# Autodesk Inventor assembly: 0905_bt_robot
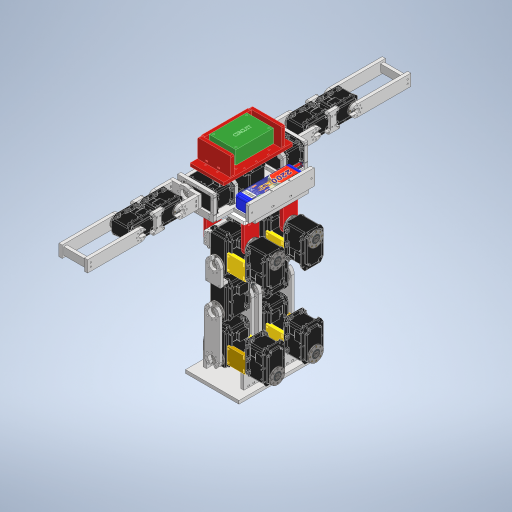
[picture p0: Inventor's stored thumbnail of the model, 512x512]
Saved by Autodesk Inventor 2024.3 (Build 283343000, 343)
## iProperties
Created: 2024-09-05
Part Number: 0905_bt_robot
Document SubType Name: Assembly
Designer: gretc
Author: gretc
## Documents named in this file (47)
- C:\Users\gretc\Desktop\inventor_part\예비인턴 격투로봇 설계 프로젝트\0905_bt_robot.iam
- C:\Users\gretc\Desktop\inventor_part\Motor_106.iam
- C:\Users\gretc\Desktop\inventor_part\Motor_64.iam
- C:\Users\gretc\Desktop\inventor_part\예비인턴 격투로봇 설계 프로젝트\_idle_adt.ipt
- C:\Users\gretc\Desktop\inventor_part\예비인턴 격투로봇 설계 프로젝트\_adle_adt_2.ipt
- C:\Users\gretc\Desktop\inventor_part\아이들러\64아이들러.iam
- C:\Users\gretc\Desktop\inventor_part\예비인턴 격투로봇 설계 프로젝트\_shim.ipt
- C:\Users\gretc\Desktop\inventor_part\예비인턴 격투로봇 설계 프로젝트\_foot.ipt
- C:\Users\gretc\Desktop\inventor_part\예비인턴 격투로봇 설계 프로젝트\_adle_adt_foot.ipt
- C:\Users\gretc\Desktop\inventor_part\예비인턴 격투로봇 설계 프로젝트\_foot_adt.ipt
- C:\Users\gretc\Desktop\inventor_part\예비인턴 격투로봇 설계 프로젝트\_108-64_adt.ipt
- C:\Users\gretc\Desktop\inventor_part\예비인턴 격투로봇 설계 프로젝트\_thigh.ipt
- C:\Users\gretc\Desktop\inventor_part\예비인턴 격투로봇 설계 프로젝트\_thigh_2.ipt
- C:\Users\gretc\Desktop\inventor_part\Motor_106_MIR.iam
- C:\Users\gretc\Desktop\inventor_part\Motor_64_MIR.iam
- C:\Users\gretc\Desktop\inventor_part\예비인턴 격투로봇 설계 프로젝트\_idle_adt_MIR.ipt
- C:\Users\gretc\Desktop\inventor_part\예비인턴 격투로봇 설계 프로젝트\_adle_adt_2_MIR.ipt
- C:\Users\gretc\Desktop\inventor_part\예비인턴 격투로봇 설계 프로젝트\_shim_MIR.ipt
- C:\Users\gretc\Desktop\inventor_part\예비인턴 격투로봇 설계 프로젝트\_foot_MIR.ipt
- C:\Users\gretc\Desktop\inventor_part\예비인턴 격투로봇 설계 프로젝트\_foot_adt_MIR.ipt
- C:\Users\gretc\Desktop\inventor_part\예비인턴 격투로봇 설계 프로젝트\_108-64_adt_MIR.ipt
- C:\Users\gretc\Desktop\inventor_part\예비인턴 격투로봇 설계 프로젝트\_thigh_MIR.ipt
- C:\Users\gretc\Desktop\inventor_part\예비인턴 격투로봇 설계 프로젝트\_thigh_2_MIR.ipt
- C:\Users\gretc\Desktop\inventor_part\아이들러\64아이들러_MIR2.iam
- C:\Users\gretc\Desktop\inventor_part\예비인턴 격투로봇 설계 프로젝트\_thigh_adt_body_MIR.ipt
- C:\Users\gretc\Desktop\inventor_part\혼\64-106Horn.ipt
- C:\Users\gretc\Desktop\inventor_part\다이나믹셀\MX-64T.ipt
- C:\Users\gretc\Desktop\inventor_part\Motor_28.iam
- C:\Users\gretc\Desktop\inventor_part\Motor_64_no_idle_ver.iam
- C:\Users\gretc\Desktop\inventor_part\예비인턴 격투로봇 설계 프로젝트\_arm_adt.ipt
- C:\Users\gretc\Desktop\inventor_part\예비인턴 격투로봇 설계 프로젝트\_armpit_adt_1.ipt
- C:\Users\gretc\Desktop\inventor_part\Power_Control_inventor\Enrichpower_2200mAh_11.1V_30C.ipt
- C:\Users\gretc\Desktop\inventor_part\예비인턴 격투로봇 설계 프로젝트\_hand_adt_ver_2_.ipt
- C:\Users\gretc\Desktop\inventor_part\예비인턴 격투로봇 설계 프로젝트\_fist_ver2_.ipt
- C:\Users\Public\Documents\Autodesk\Inventor 2024\_pelvis.ipt
- C:\Users\Public\Documents\Autodesk\Inventor 2024\_idle-pelvis_adt.ipt
- C:\Users\Public\Documents\Autodesk\Inventor 2024\_battery_adt.ipt
- C:\Users\Public\Documents\Autodesk\Inventor 2024\_battery_adt_2_.ipt
- C:\Users\Public\Documents\Autodesk\Inventor 2024\_newbody1.ipt
- C:\Users\Public\Documents\Autodesk\Inventor 2024\_face_froward_2.ipt
- C:\Users\Public\Documents\Autodesk\Inventor 2024\_body_side_ver2.ipt
- C:\Users\Public\Documents\Autodesk\Inventor 2024\head.iam
- C:\Users\Public\Documents\Autodesk\Inventor 2024\_inner.ipt
- C:\Users\Public\Documents\Autodesk\Inventor 2024\_arm_adt-ver2.ipt
- C:\Users\Public\Documents\Autodesk\Inventor 2024\_arm_pti.ipt
- C:\Users\gretc\Desktop\inventor_part\Power_Control_inventor\Circuit.ipt
- MX-106T+idle.ipt
## Components (95 placed, 45 different names)
1. Motor_106:1 [sub-assembly] — 메이트:1, 플러쉬:1, 플러쉬:2, 플러쉬:3, 플러쉬:5, 메이트:4, 메이트:6, 플러쉬:9, 플러쉬:11, 플러쉬:12, 메이트:24, 메이트:26, 메이트:29, 플러쉬:13, 삽입:3, 플러쉬:22, 메이트:38, 삽입:5, 삽입:6
2. Motor_106:2 [sub-assembly] — 플러쉬:3, 플러쉬:4, 플러쉬:5, 플러쉬:6, 메이트:3, 메이트:5, 메이트:6, 플러쉬:14, 삽입:2, 플러쉬:23, 삽입:9, 삽입:10
3. Motor_106:3 [sub-assembly] — 플러쉬:4, 플러쉬:6, 메이트:2, 메이트:5, 각도:1, 각도:2, 플러쉬:10, 메이트:8, 메이트:9, 메이트:10, 메이트:11, 삽입:11, 메이트:39, 삽입:12, 삽입:13, 삽입:22, 삽입:23
4. Motor_64:1 [sub-assembly] — 플러쉬:7, 플러쉬:8, 각도:1, 각도:2, 플러쉬:10, 메이트:8, 메이트:14, 메이트:15, 각도:5, 삽입:15
5. Motor_64:2 [sub-assembly] — 플러쉬:7, 플러쉬:8, 메이트:7, 플러쉬:9, 삽입:4, 플러쉬:20, 플러쉬:21
6. _idle_adt:1 — 플러쉬:11, 플러쉬:12, 메이트:30
7. _idle_adt:2 — 메이트:23, 메이트:25, 메이트:29
8. _adle_adt_2:1 — 플러쉬:13, 메이트:32, 삽입:1
9. 64아이들러:1 [sub-assembly] — 메이트:31, 삽입:1, 플러쉬:15, 플러쉬:16, 플러쉬:17, 메이트:33, 메이트:34, 플러쉬:18
10. _shim:1 — 플러쉬:14, 각도:3
11. _shim:2 — 삽입:2, 삽입:3
12. _foot:1 — 플러쉬:19, 플러쉬:26
13. _adle_adt_foot:1 — 플러쉬:15
14. _foot_adt:1 — 플러쉬:16, 플러쉬:17, 플러쉬:18, 각도:4
15. _foot_adt:2 — 삽입:4, 각도:4, 플러쉬:19
16. _108-64_adt:1 — 플러쉬:20, 플러쉬:21, 플러쉬:22
17. _108-64_adt:2 — 메이트:37, 삽입:5, 삽입:6
18. _thigh:1 — 플러쉬:23
19. _thigh_2:1
20. _thigh_2:2 — 삽입:7, 삽입:8
21. _thigh:2 — 삽입:7, 삽입:8, 삽입:9, 삽입:10
22. _108-64_adt:3 — 삽입:11, 메이트:39
23. _108-64_adt:4 — 삽입:12, 삽입:13
24. _foot_adt:4 — 각도:5, 삽입:15, 각도:14
25. 64아이들러:2 [sub-assembly] — 삽입:17, 메이트:40, 메이트:41, 삽입:118
26. _adle_adt_2:2 — 삽입:17, 삽입:18, 삽입:19, 삽입:20, 삽입:21
27. _idle_adt:3 — 삽입:18, 삽입:19, 삽입:22
28. _idle_adt:4 — 삽입:20, 삽입:21, 삽입:23
29. Motor_106_MIR:1 [sub-assembly] — 플러쉬:27, 플러쉬:28, 메이트:43, 메이트:44, 플러쉬:29, 플러쉬:30, 메이트:48, 플러쉬:34, 메이트:56, 메이트:57, 메이트:58, 메이트:61, 메이트:64, 메이트:65, 삽입:24, 메이트:70, 삽입:27, 삽입:28, 메이트:74
30. Motor_106_MIR:2 [sub-assembly] — 메이트:44, 플러쉬:29, 플러쉬:30, 메이트:45, 플러쉬:31, 플러쉬:32, 메이트:47, 메이트:68, 삽입:25, 메이트:75, 삽입:29, 삽입:30
31. Motor_106_MIR:3 [sub-assembly] — 메이트:45, 플러쉬:31, 플러쉬:32, 메이트:46, 메이트:49, 플러쉬:33, 각도:7, 각도:8, 메이트:51, 메이트:52, 메이트:53, 메이트:76, 삽입:33, 삽입:34, 삽입:35, 삽입:38, 삽입:41
32. Motor_64_MIR:1 [sub-assembly] — 메이트:49, 플러쉬:33, 각도:7, 각도:8, 플러쉬:35, 플러쉬:36, 메이트:54, 메이트:55, 삽입:36, 각도:11
33. Motor_64_MIR:2 [sub-assembly] — 플러쉬:34, 플러쉬:35, 플러쉬:36, 메이트:50, 삽입:26, 메이트:71, 메이트:72
34. _idle_adt_MIR:1 — 메이트:56, 메이트:57, 메이트:66
35. _idle_adt_MIR:2 — 메이트:58, 메이트:59, 메이트:62
36. _adle_adt_2_MIR:1 — 메이트:65, 메이트:67, 삽입:91
37. _shim_MIR:1 — 메이트:68, 각도:9
38. _shim_MIR:2 — 삽입:24, 삽입:25
39. _foot_MIR:1 — 메이트:69, 메이트:81
40. _foot_adt_MIR:1 — 메이트:144
41. _foot_adt_MIR:2 — 메이트:69, 삽입:26
42. _108-64_adt_MIR:1 — 메이트:70, 메이트:71, 메이트:72
43. _108-64_adt_MIR:2 — 삽입:27, 삽입:28, 메이트:73
44. _thigh_MIR:1 — 메이트:75
45. _thigh_2_MIR:1
46. _thigh_2_MIR:2 — 삽입:31, 삽입:32
47. _thigh_MIR:2 — 삽입:29, 삽입:30, 삽입:31, 삽입:32
48. _108-64_adt_MIR:3 — 메이트:76, 삽입:33
49. _108-64_adt_MIR:4 — 삽입:34, 삽입:35
50. _foot_adt_MIR:3 — 삽입:36, 각도:11, 플러쉬:102, 플러쉬:103, 플러쉬:104
51. 64아이들러_MIR2:1 [sub-assembly] — 삽입:37, 메이트:78, 메이트:79, 삽입:117
52. _adle_adt_2_MIR:2 — 삽입:37, 삽입:39, 삽입:40, 삽입:42, 삽입:43
53. _idle_adt_MIR:3 — 삽입:38, 삽입:39, 삽입:40
54. _idle_adt_MIR:4 — 삽입:41, 삽입:42, 삽입:43
55. 64아이들러:3 [sub-assembly] — 삽입:91, 메이트:143
56. MX-64T:1 — 삽입:119, 각도:15, 각도:16, 플러쉬:108, 플러쉬:109, 플러쉬:112, 플러쉬:113, 메이트:175, 메이트:176, 플러쉬:115, 플러쉬:116
57. 64-106Horn:1 — 삽입:119, 삽입:120, 플러쉬:107
58. _pelvis:1 — 플러쉬:102, 플러쉬:103, 플러쉬:104, 각도:15, 각도:16, 삽입:120, 각도:17
59. _thigh_adt_body_MIR:3 — 삽입:117, 각도:13
60. _thigh_adt_body_MIR:4 — 삽입:118, 각도:13, 각도:14
61. _idle-pelvis_adt:1 — 플러쉬:107
62. _armpit_adt_1:11 — 삽입:156, 삽입:157, 플러쉬:127
63. Motor_28:9 [sub-assembly] — 삽입:148, 삽입:149, 삽입:150, 삽입:153, 삽입:154, 삽입:155, 삽입:156, 삽입:157
64. Motor_28:10 [sub-assembly] — 삽입:144, 삽입:145, 삽입:146, 삽입:147, 삽입:151, 삽입:152, 삽입:158, 삽입:159
65. _arm_adt:9 — 삽입:150, 삽입:151, 삽입:152, 삽입:153
66. _arm_adt:10 — 삽입:146, 삽입:147, 삽입:148, 삽입:149
67. _armpit_adt_1:12 — 삽입:154, 삽입:155, 플러쉬:125, 플러쉬:126, 메이트:187, 플러쉬:132, 플러쉬:133
68. _hand_adt_ver_2_:3 — 삽입:142, 삽입:143, 삽입:144, 삽입:145
69. _hand_adt_ver_2_:4 — 삽입:158, 삽입:159
70. _fist_ver2_:3 — 삽입:142, 삽입:143
71. _arm_adt:11 — 삽입:127, 삽입:128, 삽입:129, 삽입:130
72. _fist_ver2_:4 — 삽입:140, 삽입:141
73. Motor_28:11 [sub-assembly] — 삽입:127, 삽입:129, 삽입:132, 삽입:133, 삽입:135, 삽입:136, 삽입:139
74. _arm_adt:12 — 삽입:131, 삽입:132, 삽입:133, 삽입:134
75. _hand_adt_ver_2_:5 — 삽입:139, 삽입:140, 삽입:141
76. _hand_adt_ver_2_:6 — 삽입:135, 삽입:136
77. Motor_28:12 [sub-assembly] — 삽입:128, 삽입:130, 삽입:131, 삽입:134, 삽입:137, 삽입:138, 삽입:160, 삽입:161
78. _armpit_adt_1:13 — 삽입:137, 삽입:138, 플러쉬:125, 플러쉬:126, 메이트:188, 플러쉬:130, 플러쉬:131
79. _armpit_adt_1:14 — 삽입:160, 삽입:161
80. _battery_adt_2_:1 — 삽입:125, 삽입:126, 메이트:180
81. _battery_adt:1 — 플러쉬:123, 삽입:125, 삽입:126, 메이트:179, 메이트:181, 메이트:182, 플러쉬:124
82. Enrichpower_2200mAh_11.1V_30C:1 — 플러쉬:123, 메이트:179, 메이트:180, 각도:19
83. _newbody1:1 — 플러쉬:108, 플러쉬:109, 플러쉬:112, 메이트:177, 메이트:181, 메이트:182, 플러쉬:124
84. Motor_64_no_idle_ver:1 [sub-assembly] — 플러쉬:110, 플러쉬:111, 각도:17, 플러쉬:113, 메이트:176, 플러쉬:117, 플러쉬:118, 플러쉬:119, 플러쉬:120, 메이트:183, 메이트:184, 플러쉬:128, 플러쉬:129
85. Motor_64_no_idle_ver:2 [sub-assembly] — 플러쉬:110, 플러쉬:111, 메이트:175, 메이트:177, 플러쉬:114, 삽입:121, 삽입:122, 삽입:123, 삽입:124
86. _face_froward_2:1 — 플러쉬:114, 플러쉬:115, 플러쉬:116, 플러쉬:121
87. _body_side_ver2:1 — 플러쉬:117, 플러쉬:118, 플러쉬:122, 메이트:187
88. _body_side_ver2:2 — 삽입:121, 삽입:122, 메이트:188
89. head:1 [sub-assembly] — 플러쉬:121, 각도:18, 메이트:178, 플러쉬:122, 각도:19, 삽입:162, 삽입:163
90. _inner:1 — 플러쉬:119, 플러쉬:120, 메이트:178
91. _inner:2 — 삽입:123, 삽입:124, 각도:18
92. _arm_adt-ver2:1 — 플러쉬:128
93. _arm_pti:1 — 플러쉬:129, 플러쉬:132, 플러쉬:133
94. _arm_pti:2 — 플러쉬:130, 플러쉬:131
95. Circuit:1 — 삽입:162, 삽입:163
## Relationships (289: Mate 118, Insert 89, Flush 64, Angle 18)
- 메이트:1 [Mate]: Motor_106:1
- 플러쉬:1 [Flush]: Motor_106:1
- 플러쉬:2 [Flush]: Motor_106:1
- 플러쉬:3 [Flush]: Motor_106:1 ↔ Motor_106:2
- 플러쉬:4 [Flush]: Motor_106:2 ↔ Motor_106:3
- 플러쉬:5 [Flush]: Motor_106:1 ↔ Motor_106:2
- 플러쉬:6 [Flush]: Motor_106:2 ↔ Motor_106:3
- 메이트:2 [Mate]: Motor_106:3
- 메이트:3 [Mate]: Motor_106:2
- 메이트:4 [Mate]: Motor_106:1
- 메이트:5 [Mate] (10 mm): Motor_106:2 ↔ Motor_106:3
- 메이트:6 [Mate] (10 mm): Motor_106:1 ↔ Motor_106:2
- 플러쉬:7 [Flush]: Motor_64:1 ↔ Motor_64:2
- 플러쉬:8 [Flush]: Motor_64:1 ↔ Motor_64:2
- 각도:1 [Angle] (0 deg): Motor_106:3 ↔ Motor_64:1
- 각도:2 [Angle] (0 deg): Motor_106:3 ↔ Motor_64:1
- 메이트:7 [Mate]: Motor_64:2
- 플러쉬:9 [Flush] (1.5 mm): Motor_106:1 ↔ Motor_64:2
- 플러쉬:10 [Flush] (3.1 mm): Motor_106:3 ↔ Motor_64:1
- 메이트:8 [Mate] (20 mm): Motor_106:3 ↔ Motor_64:1
- 메이트:9 [Mate]: Motor_106:3
- 메이트:10 [Mate]: Motor_106:3
- 메이트:11 [Mate]: Motor_106:3
- 메이트:12 [Mate]
- 메이트:13 [Mate]
- 메이트:14 [Mate]: Motor_64:1
- 메이트:15 [Mate]: Motor_64:1
- 메이트:16 [Mate]
- 메이트:17 [Mate]
- 메이트:18 [Mate]
- 메이트:19 [Mate]
- 메이트:20 [Mate]
- 메이트:21 [Mate]
- 메이트:22 [Mate]
- 플러쉬:11 [Flush]: Motor_106:1 ↔ _idle_adt:1
- 플러쉬:12 [Flush]: Motor_106:1 ↔ _idle_adt:1
- 메이트:23 [Mate]: _idle_adt:2
- 메이트:24 [Mate]: Motor_106:1
- 메이트:25 [Mate]: _idle_adt:2
- 메이트:26 [Mate]: Motor_106:1
- 메이트:27 [Mate]
- 메이트:28 [Mate]
- 메이트:29 [Mate]: Motor_106:1 ↔ _idle_adt:2
- 플러쉬:13 [Flush]: Motor_106:1 ↔ _adle_adt_2:1
- 메이트:30 [Mate]: _idle_adt:1
- 메이트:31 [Mate]: 64아이들러:1
- 메이트:32 [Mate]: _adle_adt_2:1
- 삽입:1 [Insert] (0.5 mm): _adle_adt_2:1 ↔ 64아이들러:1
- 플러쉬:14 [Flush]: Motor_106:2 ↔ _shim:1
- 삽입:2 [Insert]: Motor_106:2 ↔ _shim:2
- 삽입:3 [Insert]: Motor_106:1 ↔ _shim:2
- 플러쉬:15 [Flush]: 64아이들러:1 ↔ _adle_adt_foot:1
- 플러쉬:16 [Flush]: 64아이들러:1 ↔ _foot_adt:1
- 플러쉬:17 [Flush]: 64아이들러:1 ↔ _foot_adt:1
- 메이트:33 [Mate]: 64아이들러:1
- 메이트:34 [Mate]: 64아이들러:1
- 메이트:35 [Mate]
- 메이트:36 [Mate]
- 각도:3 [Angle] (90 deg): _shim:1
- 플러쉬:18 [Flush]: 64아이들러:1 ↔ _foot_adt:1
- 삽입:4 [Insert]: Motor_64:2 ↔ _foot_adt:2
- 각도:4 [Angle] (0 deg): _foot_adt:1 ↔ _foot_adt:2
- 플러쉬:19 [Flush]: _foot:1 ↔ _foot_adt:2
- 플러쉬:20 [Flush]: Motor_64:2 ↔ _108-64_adt:1
- 플러쉬:21 [Flush]: Motor_64:2 ↔ _108-64_adt:1
- 플러쉬:22 [Flush]: Motor_106:1 ↔ _108-64_adt:1
- 메이트:37 [Mate]: _108-64_adt:2
- 메이트:38 [Mate]: Motor_106:1
- 삽입:5 [Insert]: Motor_106:1 ↔ _108-64_adt:2
- 삽입:6 [Insert]: Motor_106:1 ↔ _108-64_adt:2
- 플러쉬:23 [Flush]: Motor_106:2 ↔ _thigh:1
- 삽입:7 [Insert]: _thigh_2:2 ↔ _thigh:2
- 삽입:8 [Insert]: _thigh_2:2 ↔ _thigh:2
- 삽입:9 [Insert]: Motor_106:2 ↔ _thigh:2
- 삽입:10 [Insert]: Motor_106:2 ↔ _thigh:2
- 삽입:11 [Insert]: Motor_106:3 ↔ _108-64_adt:3
- 메이트:39 [Mate]: Motor_106:3 ↔ _108-64_adt:3
- 삽입:12 [Insert]: Motor_106:3 ↔ _108-64_adt:4
- 삽입:13 [Insert]: Motor_106:3 ↔ _108-64_adt:4
- 각도:5 [Angle] (0 deg): Motor_64:1 ↔ _foot_adt:4
- 삽입:15 [Insert] (0.5 mm): Motor_64:1 ↔ _foot_adt:4
- 삽입:17 [Insert]: 64아이들러:2 ↔ _adle_adt_2:2
- 삽입:18 [Insert]: _adle_adt_2:2 ↔ _idle_adt:3
- 삽입:19 [Insert]: _adle_adt_2:2 ↔ _idle_adt:3
- 삽입:20 [Insert]: _adle_adt_2:2 ↔ _idle_adt:4
- 삽입:21 [Insert]: _adle_adt_2:2 ↔ _idle_adt:4
- 삽입:22 [Insert]: Motor_106:3 ↔ _idle_adt:3
- 삽입:23 [Insert]: Motor_106:3 ↔ _idle_adt:4
- 메이트:40 [Mate]: 64아이들러:2
- 메이트:41 [Mate]: 64아이들러:2
- 각도:6 [Angle] (0 deg)
- 플러쉬:26 [Flush] (1 mm): _foot:1
- 플러쉬:27 [Flush]: Motor_106_MIR:1
- 플러쉬:28 [Flush]: Motor_106_MIR:1
- 메이트:43 [Mate]: Motor_106_MIR:1
- 메이트:44 [Mate] (10 mm): Motor_106_MIR:1 ↔ Motor_106_MIR:2
- 플러쉬:29 [Flush]: Motor_106_MIR:1 ↔ Motor_106_MIR:2
- 플러쉬:30 [Flush]: Motor_106_MIR:1 ↔ Motor_106_MIR:2
- 메이트:45 [Mate] (10 mm): Motor_106_MIR:2 ↔ Motor_106_MIR:3
- 플러쉬:31 [Flush]: Motor_106_MIR:2 ↔ Motor_106_MIR:3
- 플러쉬:32 [Flush]: Motor_106_MIR:2 ↔ Motor_106_MIR:3
- 메이트:46 [Mate]: Motor_106_MIR:3
- 메이트:47 [Mate]: Motor_106_MIR:2
- 메이트:48 [Mate]: Motor_106_MIR:1
- 메이트:49 [Mate] (20 mm): Motor_106_MIR:3 ↔ Motor_64_MIR:1
- 플러쉬:33 [Flush] (3.1 mm): Motor_106_MIR:3 ↔ Motor_64_MIR:1
- 각도:7 [Angle] (0 deg): Motor_106_MIR:3 ↔ Motor_64_MIR:1
- 각도:8 [Angle] (0 deg): Motor_106_MIR:3 ↔ Motor_64_MIR:1
- 플러쉬:34 [Flush] (1.5 mm): Motor_106_MIR:1 ↔ Motor_64_MIR:2
- 플러쉬:35 [Flush]: Motor_64_MIR:1 ↔ Motor_64_MIR:2
- 플러쉬:36 [Flush]: Motor_64_MIR:1 ↔ Motor_64_MIR:2
- 메이트:50 [Mate]: Motor_64_MIR:2
- 메이트:51 [Mate]: Motor_106_MIR:3
- 메이트:52 [Mate]: Motor_106_MIR:3
- 메이트:53 [Mate]: Motor_106_MIR:3
- 메이트:54 [Mate]: Motor_64_MIR:1
- 메이트:55 [Mate]: Motor_64_MIR:1
- 메이트:56 [Mate]: Motor_106_MIR:1 ↔ _idle_adt_MIR:1
- 메이트:57 [Mate]: Motor_106_MIR:1 ↔ _idle_adt_MIR:1
- 메이트:58 [Mate]: Motor_106_MIR:1 ↔ _idle_adt_MIR:2
- 메이트:59 [Mate]: _idle_adt_MIR:2
- 메이트:60 [Mate]
- 메이트:61 [Mate]: Motor_106_MIR:1
- 메이트:62 [Mate]: _idle_adt_MIR:2
- 메이트:63 [Mate]
- 메이트:64 [Mate]: Motor_106_MIR:1
- 메이트:65 [Mate]: Motor_106_MIR:1 ↔ _adle_adt_2_MIR:1
- 메이트:66 [Mate]: _idle_adt_MIR:1
- 메이트:67 [Mate]: _adle_adt_2_MIR:1
- 메이트:68 [Mate]: Motor_106_MIR:2 ↔ _shim_MIR:1
- 삽입:24 [Insert]: Motor_106_MIR:1 ↔ _shim_MIR:2
- 삽입:25 [Insert]: Motor_106_MIR:2 ↔ _shim_MIR:2
- 각도:9 [Angle] (90 deg): _shim_MIR:1
- 메이트:69 [Mate]: _foot_MIR:1 ↔ _foot_adt_MIR:2
- 삽입:26 [Insert]: Motor_64_MIR:2 ↔ _foot_adt_MIR:2
- 메이트:70 [Mate]: Motor_106_MIR:1 ↔ _108-64_adt_MIR:1
- 메이트:71 [Mate]: Motor_64_MIR:2 ↔ _108-64_adt_MIR:1
- 메이트:72 [Mate]: Motor_64_MIR:2 ↔ _108-64_adt_MIR:1
- 삽입:27 [Insert]: Motor_106_MIR:1 ↔ _108-64_adt_MIR:2
- 삽입:28 [Insert]: Motor_106_MIR:1 ↔ _108-64_adt_MIR:2
- 메이트:73 [Mate]: _108-64_adt_MIR:2
- 메이트:74 [Mate]: Motor_106_MIR:1
- 메이트:75 [Mate]: Motor_106_MIR:2 ↔ _thigh_MIR:1
- 삽입:29 [Insert]: Motor_106_MIR:2 ↔ _thigh_MIR:2
- 삽입:30 [Insert]: Motor_106_MIR:2 ↔ _thigh_MIR:2
- 삽입:31 [Insert]: _thigh_2_MIR:2 ↔ _thigh_MIR:2
- 삽입:32 [Insert]: _thigh_2_MIR:2 ↔ _thigh_MIR:2
- 메이트:76 [Mate]: Motor_106_MIR:3 ↔ _108-64_adt_MIR:3
- 삽입:33 [Insert]: Motor_106_MIR:3 ↔ _108-64_adt_MIR:3
- 삽입:34 [Insert]: Motor_106_MIR:3 ↔ _108-64_adt_MIR:4
- 삽입:35 [Insert]: Motor_106_MIR:3 ↔ _108-64_adt_MIR:4
- 삽입:36 [Insert] (0.5 mm): Motor_64_MIR:1 ↔ _foot_adt_MIR:3
- 각도:11 [Angle] (0 deg): Motor_64_MIR:1 ↔ _foot_adt_MIR:3
- 삽입:37 [Insert]: 64아이들러_MIR2:1 ↔ _adle_adt_2_MIR:2
- 삽입:38 [Insert]: Motor_106_MIR:3 ↔ _idle_adt_MIR:3
- 삽입:39 [Insert]: _adle_adt_2_MIR:2 ↔ _idle_adt_MIR:3
- 삽입:40 [Insert]: _adle_adt_2_MIR:2 ↔ _idle_adt_MIR:3
- 삽입:41 [Insert]: Motor_106_MIR:3 ↔ _idle_adt_MIR:4
- 삽입:42 [Insert]: _adle_adt_2_MIR:2 ↔ _idle_adt_MIR:4
- 삽입:43 [Insert]: _adle_adt_2_MIR:2 ↔ _idle_adt_MIR:4
- 메이트:78 [Mate]: 64아이들러_MIR2:1
- 메이트:79 [Mate]: 64아이들러_MIR2:1
- 각도:12 [Angle] (0 deg)
- 메이트:81 [Mate] (1 mm): _foot_MIR:1
- 메이트:85 [Mate]
- 메이트:86 [Mate]
- 메이트:106 [Mate]
- 메이트:107 [Mate]
- 메이트:108 [Mate]
- 메이트:109 [Mate]
- 메이트:110 [Mate]
- 메이트:111 [Mate]
- 메이트:112 [Mate]
- 메이트:113 [Mate]
- 메이트:118 [Mate]
- 메이트:119 [Mate]
- 메이트:120 [Mate]
- 메이트:121 [Mate]
- 메이트:142 [Mate]
- 삽입:91 [Insert] (0.5 mm): _adle_adt_2_MIR:1 ↔ 64아이들러:3
- 메이트:143 [Mate]: 64아이들러:3
- 메이트:144 [Mate]: _foot_adt_MIR:1
- 메이트:145 [Mate]
- 메이트:148 [Mate]
- 메이트:151 [Mate]
- 플러쉬:102 [Flush]: _foot_adt_MIR:3 ↔ _pelvis:1
- 플러쉬:103 [Flush]: _foot_adt_MIR:3 ↔ _pelvis:1
- 삽입:117 [Insert]: 64아이들러_MIR2:1 ↔ _thigh_adt_body_MIR:3
- 삽입:118 [Insert]: 64아이들러:2 ↔ _thigh_adt_body_MIR:4
- 각도:13 [Angle] (0 deg): _thigh_adt_body_MIR:3 ↔ _thigh_adt_body_MIR:4
- 각도:14 [Angle] (0 deg): _foot_adt:4 ↔ _thigh_adt_body_MIR:4
- 플러쉬:104 [Flush]: _foot_adt_MIR:3 ↔ _pelvis:1
- 삽입:119 [Insert] (0.5 mm): MX-64T:1 ↔ 64-106Horn:1
- 각도:15 [Angle] (0 deg): MX-64T:1 ↔ _pelvis:1
- 각도:16 [Angle] (0 deg): MX-64T:1 ↔ _pelvis:1
- 삽입:120 [Insert] (6 mm): 64-106Horn:1 ↔ _pelvis:1
- 플러쉬:107 [Flush]: 64-106Horn:1 ↔ _idle-pelvis_adt:1
- 메이트:161 [Mate]
- 메이트:164 [Mate]
- 메이트:166 [Mate]
- 메이트:169 [Mate]
- 메이트:173 [Mate]
- 메이트:174 [Mate]
- 플러쉬:108 [Flush]: MX-64T:1 ↔ _newbody1:1
- 플러쉬:109 [Flush]: MX-64T:1 ↔ _newbody1:1
- 플러쉬:110 [Flush]: Motor_64_no_idle_ver:1 ↔ Motor_64_no_idle_ver:2
- 플러쉬:111 [Flush]: Motor_64_no_idle_ver:1 ↔ Motor_64_no_idle_ver:2
- 각도:17 [Angle] (0 deg): _pelvis:1 ↔ Motor_64_no_idle_ver:1
- 플러쉬:112 [Flush]: MX-64T:1 ↔ _newbody1:1
- 플러쉬:113 [Flush]: MX-64T:1 ↔ Motor_64_no_idle_ver:1
- 메이트:175 [Mate] (30 mm): MX-64T:1 ↔ Motor_64_no_idle_ver:2
- 메이트:176 [Mate] (30 mm): MX-64T:1 ↔ Motor_64_no_idle_ver:1
- 메이트:177 [Mate]: _newbody1:1 ↔ Motor_64_no_idle_ver:2
- 플러쉬:114 [Flush]: Motor_64_no_idle_ver:2 ↔ _face_froward_2:1
- 플러쉬:115 [Flush]: MX-64T:1 ↔ _face_froward_2:1
- 플러쉬:116 [Flush]: MX-64T:1 ↔ _face_froward_2:1
- 플러쉬:117 [Flush]: Motor_64_no_idle_ver:1 ↔ _body_side_ver2:1
- 플러쉬:118 [Flush]: Motor_64_no_idle_ver:1 ↔ _body_side_ver2:1
- 삽입:121 [Insert]: Motor_64_no_idle_ver:2 ↔ _body_side_ver2:2
- 삽입:122 [Insert]: Motor_64_no_idle_ver:2 ↔ _body_side_ver2:2
- 플러쉬:119 [Flush]: Motor_64_no_idle_ver:1 ↔ _inner:1
- 플러쉬:120 [Flush]: Motor_64_no_idle_ver:1 ↔ _inner:1
- 삽입:123 [Insert]: Motor_64_no_idle_ver:2 ↔ _inner:2
- 삽입:124 [Insert]: Motor_64_no_idle_ver:2 ↔ _inner:2
- 플러쉬:121 [Flush]: _face_froward_2:1 ↔ head:1
- 각도:18 [Angle] (0 deg): head:1 ↔ _inner:2
- 메이트:178 [Mate]: head:1 ↔ _inner:1
- 플러쉬:122 [Flush] (37.4 mm): _body_side_ver2:1 ↔ head:1
- 플러쉬:123 [Flush]: _battery_adt:1 ↔ Enrichpower_2200mAh_11.1V_30C:1
- 삽입:125 [Insert]: _battery_adt_2_:1 ↔ _battery_adt:1
- 삽입:126 [Insert]: _battery_adt_2_:1 ↔ _battery_adt:1
- 메이트:179 [Mate]: _battery_adt:1 ↔ Enrichpower_2200mAh_11.1V_30C:1
- 메이트:180 [Mate]: _battery_adt_2_:1 ↔ Enrichpower_2200mAh_11.1V_30C:1
- 메이트:181 [Mate]: _battery_adt:1 ↔ _newbody1:1
- 메이트:182 [Mate]: _battery_adt:1 ↔ _newbody1:1
- 각도:19 [Angle] (0 deg): Enrichpower_2200mAh_11.1V_30C:1 ↔ head:1
- 플러쉬:124 [Flush]: _battery_adt:1 ↔ _newbody1:1
- 삽입:127 [Insert]: _arm_adt:11 ↔ Motor_28:11
- 삽입:128 [Insert]: _arm_adt:11 ↔ Motor_28:12
- 삽입:129 [Insert]: _arm_adt:11 ↔ Motor_28:11
- 삽입:130 [Insert]: _arm_adt:11 ↔ Motor_28:12
- 삽입:131 [Insert]: _arm_adt:12 ↔ Motor_28:12
- 삽입:132 [Insert]: Motor_28:11 ↔ _arm_adt:12
- 삽입:133 [Insert]: Motor_28:11 ↔ _arm_adt:12
- 삽입:134 [Insert]: _arm_adt:12 ↔ Motor_28:12
- 삽입:135 [Insert]: Motor_28:11 ↔ _hand_adt_ver_2_:6
- 삽입:136 [Insert]: Motor_28:11 ↔ _hand_adt_ver_2_:6
- 삽입:137 [Insert]: Motor_28:12 ↔ _armpit_adt_1:13
- 삽입:138 [Insert]: Motor_28:12 ↔ _armpit_adt_1:13
- 삽입:139 [Insert]: Motor_28:11 ↔ _hand_adt_ver_2_:5
- 삽입:140 [Insert]: _fist_ver2_:4 ↔ _hand_adt_ver_2_:5
- 삽입:141 [Insert]: _fist_ver2_:4 ↔ _hand_adt_ver_2_:5
- 삽입:142 [Insert]: _hand_adt_ver_2_:3 ↔ _fist_ver2_:3
- 삽입:143 [Insert]: _hand_adt_ver_2_:3 ↔ _fist_ver2_:3
- 삽입:144 [Insert]: Motor_28:10 ↔ _hand_adt_ver_2_:3
- 삽입:145 [Insert]: Motor_28:10 ↔ _hand_adt_ver_2_:3
- 삽입:146 [Insert]: Motor_28:10 ↔ _arm_adt:10
- 삽입:147 [Insert]: Motor_28:10 ↔ _arm_adt:10
- 삽입:148 [Insert]: Motor_28:9 ↔ _arm_adt:10
- 삽입:149 [Insert]: Motor_28:9 ↔ _arm_adt:10
- 삽입:150 [Insert]: Motor_28:9 ↔ _arm_adt:9
- 삽입:151 [Insert]: Motor_28:10 ↔ _arm_adt:9
- 삽입:152 [Insert]: Motor_28:10 ↔ _arm_adt:9
- 삽입:153 [Insert]: Motor_28:9 ↔ _arm_adt:9
- 삽입:154 [Insert]: Motor_28:9 ↔ _armpit_adt_1:12
- 삽입:155 [Insert]: Motor_28:9 ↔ _armpit_adt_1:12
- 삽입:156 [Insert]: _armpit_adt_1:11 ↔ Motor_28:9
- 삽입:157 [Insert]: _armpit_adt_1:11 ↔ Motor_28:9
- 삽입:158 [Insert]: Motor_28:10 ↔ _hand_adt_ver_2_:4
- 삽입:159 [Insert]: Motor_28:10 ↔ _hand_adt_ver_2_:4
- 삽입:160 [Insert]: Motor_28:12 ↔ _armpit_adt_1:14
- 삽입:161 [Insert]: Motor_28:12 ↔ _armpit_adt_1:14
- 플러쉬:125 [Flush]: _armpit_adt_1:12 ↔ _armpit_adt_1:13
- 플러쉬:126 [Flush]: _armpit_adt_1:12 ↔ _armpit_adt_1:13
- 메이트:183 [Mate]: Motor_64_no_idle_ver:1
- 메이트:184 [Mate]: Motor_64_no_idle_ver:1
- 메이트:185 [Mate]
- 메이트:186 [Mate]
- 플러쉬:127 [Flush] (26.75 mm): _armpit_adt_1:11
- 플러쉬:128 [Flush]: Motor_64_no_idle_ver:1 ↔ _arm_adt-ver2:1
- 메이트:187 [Mate] (7 mm): _armpit_adt_1:12 ↔ _body_side_ver2:1
- 메이트:188 [Mate] (7 mm): _armpit_adt_1:13 ↔ _body_side_ver2:2
- 플러쉬:129 [Flush]: Motor_64_no_idle_ver:1 ↔ _arm_pti:1
- 플러쉬:130 [Flush]: _armpit_adt_1:13 ↔ _arm_pti:2
- 플러쉬:131 [Flush]: _armpit_adt_1:13 ↔ _arm_pti:2
- 플러쉬:132 [Flush]: _armpit_adt_1:12 ↔ _arm_pti:1
- 플러쉬:133 [Flush]: _armpit_adt_1:12 ↔ _arm_pti:1
- 삽입:162 [Insert] (10 mm): head:1 ↔ Circuit:1
- 삽입:163 [Insert] (10 mm): head:1 ↔ Circuit:1
